# Autodesk Inventor assembly: Sheep
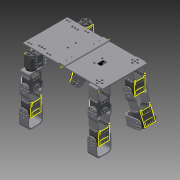
[picture p0: Inventor's stored thumbnail of the model, 180x180]
Saved by Autodesk Inventor 2014 SP1 (Build 180222100, 222)
## iProperties
Created: 2014-04-23
Part Number: Sheep
Document SubType Name: Assembly
Designer: david
Author: david
## Documents named in this file (12)
- C:\Users\asus\Documents\GitHub\SheepWarrior\Autodesk\V2\Sheep\Sheep.iam
- C:\Users\asus\Documents\GitHub\SheepWarrior\Autodesk\V2\Sheep\Equerre.ipt
- C:\Users\asus\Documents\GitHub\SheepWarrior\Autodesk\V2\XL320\src\Motor.iam
- C:\Users\asus\Documents\GitHub\SheepWarrior\Autodesk\V2\XL320\src\Pantilt.ipt
- C:\Users\asus\Documents\GitHub\SheepWarrior\Autodesk\V2\XL320\src\ArmToBottom.ipt
- C:\Users\asus\Documents\GitHub\SheepWarrior\Autodesk\V2\Sheep\Board.ipt
- C:\Users\asus\Documents\GitHub\SheepWarrior\Autodesk\V2\Sheep\BackLegUpperBone.ipt
- C:\Users\asus\Documents\GitHub\SheepWarrior\Autodesk\V2\Sheep\BackLegMiddleBone.ipt
- C:\Users\asus\Documents\GitHub\SheepWarrior\Autodesk\V2\Sheep\BackFeet.ipt
- C:\Users\asus\Documents\GitHub\SheepWarrior\Autodesk\V2\Sheep\FrontFeet.ipt
- C:\Users\asus\Documents\GitHub\SheepWarrior\Autodesk\V2\Sheep\BodyBack.ipt
- C:\Users\asus\Documents\GitHub\SheepWarrior\Autodesk\V2\Sheep\BodyFront.ipt
## Components (33 placed, 10 different names)
1. Equerre:1 — Mate:115, Mate:133, Mate:134
2. Equerre:2 — Mate:112, Mate:135, Mate:136
3. Motor:1 [sub-assembly] — Mate:17, Rotational:1, Mate:106, Mate:107, Mate:108, Mate:109, Mate:110, Mate:111, Mate:124, Mate:125, Mate:126
4. Pantilt:1 — Mate:17, Rotational:1, Mate:18, Mate:19, Mate:20
5. Motor:2 [sub-assembly] — Mate:18, Mate:19, Mate:20, Mate:21, Mate:24, Rotational:2, Rotational:3
6. ArmToBottom:1 — Mate:21, Rotational:3, Mate:25, Mate:26, Mate:27
7. ArmToBottom:2 — Mate:24, Rotational:2, Mate:28
8. Motor:3 [sub-assembly] — Mate:25, Mate:26, Mate:27, Mate:28, Mate:102, Rotational:20
9. Motor:4 [sub-assembly] — Mate:85, Mate:86, Mate:87, Mate:91, Mate:92, Mate:93, Rotational:17
10. Motor:5 [sub-assembly] — Mate:94, Mate:95, Mate:97, Mate:99, Mate:100
11. Motor:6 [sub-assembly] — Mate:79, Mate:80, Mate:81, Mate:88, Rotational:15, Rotational:16
12. Motor:7 [sub-assembly] — Mate:89, Mate:90, Mate:96, Mate:98, Rotational:18
13. Equerre:3 — Mate:109, Mate:110, Mate:111
14. Equerre:4 — Mate:106, Mate:107, Mate:108
15. Motor:8 [sub-assembly] — Mate:63, Rotational:11, Mate:112, Mate:115, Mate:121, Mate:122, Mate:123
16. Motor:9 [sub-assembly] — Mate:69, Mate:70, Mate:71, Mate:101, Rotational:19
17. Motor:10 [sub-assembly] — Mate:64, Mate:65, Mate:66, Mate:67, Rotational:12, Mate:68, Rotational:13
18. Pantilt:4 — Mate:63, Rotational:11, Mate:64, Mate:65, Mate:66
19. ArmToBottom:7 — Mate:67, Rotational:12, Mate:69, Mate:70
20. ArmToBottom:8 — Mate:68, Rotational:13, Mate:71
21. Board:1 — Mate:118, Mate:119, Mate:120
22. BackLegUpperBone:1 — Mate:79, Mate:80, Mate:81, Mate:127, Mate:128, Mate:129
23. BackLegUpperBone:2 — Mate:85, Mate:86, Mate:87, Mate:130, Mate:131, Mate:132
24. BackLegMiddleBone:1 — Rotational:16, Mate:90
25. BackLegMiddleBone:2 — Mate:88, Rotational:15, Mate:89, Mate:96
26. BackLegMiddleBone:3 — Mate:91, Mate:92, Mate:95
27. BackLegMiddleBone:4 — Mate:93, Rotational:17, Mate:94, Mate:97
28. BackFeet:1 — Mate:98, Rotational:18
29. BackFeet:2 — Mate:99, Mate:100
30. FrontFeet:1 — Mate:101, Rotational:19
31. FrontFeet:2 — Mate:102, Rotational:20
32. Body:2 — Mate:103, Mate:104, Mate:105, Mate:120, Mate:127, Mate:128, Mate:129, Mate:130, Mate:131, Mate:132
33. Body:3 — Mate:103, Mate:104, Mate:105, Mate:118, Mate:119, Mate:121, Mate:122, Mate:123, Mate:124, Mate:125, Mate:126, Mate:133, Mate:134, Mate:135, Mate:136
## Relationships (82: Mate 70, RevoluteJoint 12)
- Mate:17: Motor:1 ↔ Pantilt:1
- Rotational:1 [RevoluteJoint]: Motor:1 ↔ Pantilt:1
- Mate:18: Pantilt:1 ↔ Motor:2
- Mate:19: Pantilt:1 ↔ Motor:2
- Mate:20: Pantilt:1 ↔ Motor:2
- Mate:21: Motor:2 ↔ ArmToBottom:1
- Mate:24: Motor:2 ↔ ArmToBottom:2
- Rotational:2 [RevoluteJoint]: Motor:2 ↔ ArmToBottom:2
- Rotational:3 [RevoluteJoint]: Motor:2 ↔ ArmToBottom:1
- Mate:25: ArmToBottom:1 ↔ Motor:3
- Mate:26: ArmToBottom:1 ↔ Motor:3
- Mate:27: ArmToBottom:1 ↔ Motor:3
- Mate:28: ArmToBottom:2 ↔ Motor:3
- Mate:63: Motor:8 ↔ Pantilt:4
- Rotational:11 [RevoluteJoint]: Motor:8 ↔ Pantilt:4
- Mate:64: Motor:10 ↔ Pantilt:4
- Mate:65: Motor:10 ↔ Pantilt:4
- Mate:66: Motor:10 ↔ Pantilt:4
- Mate:67: Motor:10 ↔ ArmToBottom:7
- Rotational:12 [RevoluteJoint]: Motor:10 ↔ ArmToBottom:7
- Mate:68: Motor:10 ↔ ArmToBottom:8
- Rotational:13 [RevoluteJoint]: Motor:10 ↔ ArmToBottom:8
- Mate:69: Motor:9 ↔ ArmToBottom:7
- Mate:70: Motor:9 ↔ ArmToBottom:7
- Mate:71: Motor:9 ↔ ArmToBottom:8
- Mate:79: Motor:6 ↔ BackLegUpperBone:1
- Mate:80: Motor:6 ↔ BackLegUpperBone:1
- Mate:81: Motor:6 ↔ BackLegUpperBone:1
- Mate:85: Motor:4 ↔ BackLegUpperBone:2
- Mate:86: Motor:4 ↔ BackLegUpperBone:2
- Mate:87: Motor:4 ↔ BackLegUpperBone:2
- Mate:88: Motor:6 ↔ BackLegMiddleBone:2
- Rotational:15 [RevoluteJoint]: Motor:6 ↔ BackLegMiddleBone:2
- Rotational:16 [RevoluteJoint]: Motor:6 ↔ BackLegMiddleBone:1
- Mate:89: Motor:7 ↔ BackLegMiddleBone:2
- Mate:90: Motor:7 ↔ BackLegMiddleBone:1
- Mate:91: Motor:4 ↔ BackLegMiddleBone:3
- Mate:92: Motor:4 ↔ BackLegMiddleBone:3
- Mate:93: Motor:4 ↔ BackLegMiddleBone:4
- Rotational:17 [RevoluteJoint]: Motor:4 ↔ BackLegMiddleBone:4
- Mate:94: Motor:5 ↔ BackLegMiddleBone:4
- Mate:95: Motor:5 ↔ BackLegMiddleBone:3
- Mate:96: Motor:7 ↔ BackLegMiddleBone:2
- Mate:97: Motor:5 ↔ BackLegMiddleBone:4
- Mate:98: Motor:7 ↔ BackFeet:1
- Rotational:18 [RevoluteJoint]: Motor:7 ↔ BackFeet:1
- Mate:99: Motor:5 ↔ BackFeet:2
- Mate:100: Motor:5 ↔ BackFeet:2
- Mate:101: Motor:9 ↔ FrontFeet:1
- Mate:102: Motor:3 ↔ FrontFeet:2
- Rotational:19 [RevoluteJoint]: Motor:9 ↔ FrontFeet:1
- Rotational:20 [RevoluteJoint]: Motor:3 ↔ FrontFeet:2
- Mate:103: Body:2 ↔ Body:3
- Mate:104: Body:2 ↔ Body:3
- Mate:105: Body:2 ↔ Body:3
- Mate:106: Motor:1 ↔ Equerre:4
- Mate:107: Motor:1 ↔ Equerre:4
- Mate:108: Motor:1 ↔ Equerre:4
- Mate:109: Motor:1 ↔ Equerre:3
- Mate:110: Motor:1 ↔ Equerre:3
- Mate:111: Motor:1 ↔ Equerre:3
- Mate:112: Equerre:2 ↔ Motor:8
- Mate:115: Equerre:1 ↔ Motor:8
- Mate:118: Board:1 ↔ Body:3
- Mate:119: Board:1 ↔ Body:3
- Mate:120: Board:1 ↔ Body:2
- Mate:121: Motor:8 ↔ Body:3
- Mate:122: Motor:8 ↔ Body:3
- Mate:123: Motor:8 ↔ Body:3
- Mate:124: Motor:1 ↔ Body:3
- Mate:125: Motor:1 ↔ Body:3
- Mate:126: Motor:1 ↔ Body:3
- Mate:127: BackLegUpperBone:1 ↔ Body:2
- Mate:128: BackLegUpperBone:1 ↔ Body:2
- Mate:129: BackLegUpperBone:1 ↔ Body:2
- Mate:130: BackLegUpperBone:2 ↔ Body:2
- Mate:131: BackLegUpperBone:2 ↔ Body:2
- Mate:132: BackLegUpperBone:2 ↔ Body:2
- Mate:133: Equerre:1 ↔ Body:3
- Mate:134: Equerre:1 ↔ Body:3
- Mate:135: Equerre:2 ↔ Body:3
- Mate:136: Equerre:2 ↔ Body:3
